# Autodesk Inventor assembly: controller
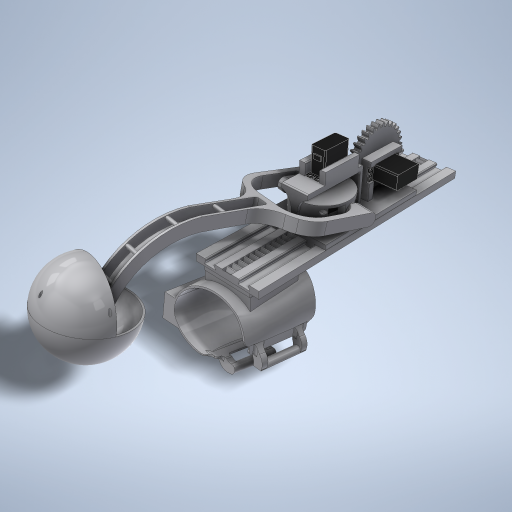
[picture p0: Inventor's stored thumbnail of the model, 512x512]
Saved by Autodesk Inventor 2023 (Build 270158000, 158)
## iProperties
Created: 2024-09-29
Part Number: controller
Document SubType Name: Assembly
Designer: dennis
Author: dennis
## Documents named in this file (15)
- E:\files\controller_v2\final\controller_backup.iam
- E:\files\controller_v2\final\bangle.ipt
- E:\files\controller_v2\final\bangle_ rail_connector.ipt
- E:\files\controller_v2\final\rail.ipt
- rail.ipt
- E:\files\controller_v2\final\carriage.ipt
- E:\files\controller_v2\final\servo_alzrc_ds452mg.ipt
- E:\files\controller_v2\final\servo_horn.ipt
- E:\files\controller_v2\final\gear.ipt
- E:\files\controller_v2\final\ballbearing_servo_mount_swing_axis.ipt
- E:\files\controller_v2\final\servo_mount_swing_axis.ipt
- E:\files\controller_v2\final\ballbearing_pivot_axis.ipt
- E:\files\controller_v2\final\lever.ipt
- E:\files\controller_v2\final\end_effector_halfball.ipt
- E:\files\controller_v2\final\end_effector_quarterball.ipt
## Components (17 placed, 13 different names)
1. bangle_ rail_connector:1 — Slider:1, Rigid:1
2. bangle:1 — Slider:1
3. rail:1 — Rigid:1, Slider:2
4. carriage:1 — Slider:2, Rigid:2, Rotation/Translation:1, Rotation/Translation:2, Rotational:3, Rigid:3
5. servo_alzrc_ds452mg:1 — Rigid:2, Rotational:1
6. servo_horn:1 — Rotational:1, Rotation/Translation:1, Rotational:2
7. gear:1 — Rotational:2, Rotation/Translation:2
8. ballbearing_servo_mount_swing_axis:1 — Rotational:3
9. servo_alzrc_ds452mg:2 — Rigid:3, Rotational:4
10. servo_horn:2 — Rotational:4, Rigid:6
11. servo_mount_swing_axis:1 — Rigid:6, Rigid:7, Rigid:8
12. ballbearing_pivot_axis:1 — Rigid:7
13. servo_alzrc_ds452mg:3 — Rigid:8, Rotational:5
14. servo_horn:3 — Rotational:5, Rigid:9
15. lever:1 — Rigid:9, Rigid:10
16. end_effector_quarterball:1 — Rigid:10, Rigid:11
17. end_effector_halfball:1 — Rigid:11
## Relationships (18: WeldJoint 9, RevoluteJoint 5, TranslationJoint 2, RelateRotateTranslate 2)
- Slider:1 [TranslationJoint]: bangle_ rail_connector:1 ↔ bangle:1
- Rigid:1 [WeldJoint]: bangle_ rail_connector:1 ↔ rail:1
- Slider:2 [TranslationJoint]: rail:1 ↔ carriage:1
- Rigid:2 [WeldJoint]: carriage:1 ↔ servo_alzrc_ds452mg:1
- Rotational:1 [RevoluteJoint]: servo_alzrc_ds452mg:1 ↔ servo_horn:1
- Rotation/Translation:1 [RelateRotateTranslate] (160 mm): carriage:1 ↔ servo_horn:1
- Rotational:2 [RevoluteJoint]: servo_horn:1 ↔ gear:1
- Rotation/Translation:2 [RelateRotateTranslate] (160 mm): carriage:1 ↔ gear:1
- Rotational:3 [RevoluteJoint]: carriage:1 ↔ ballbearing_servo_mount_swing_axis:1
- Rigid:3 [WeldJoint]: carriage:1 ↔ servo_alzrc_ds452mg:2
- Rotational:4 [RevoluteJoint]: servo_alzrc_ds452mg:2 ↔ servo_horn:2
- Rigid:6 [WeldJoint]: servo_horn:2 ↔ servo_mount_swing_axis:1
- Rigid:7 [WeldJoint]: servo_mount_swing_axis:1 ↔ ballbearing_pivot_axis:1
- Rigid:8 [WeldJoint]: servo_mount_swing_axis:1 ↔ servo_alzrc_ds452mg:3
- Rotational:5 [RevoluteJoint]: servo_alzrc_ds452mg:3 ↔ servo_horn:3
- Rigid:9 [WeldJoint]: servo_horn:3 ↔ lever:1
- Rigid:10 [WeldJoint]: lever:1 ↔ end_effector_quarterball:1
- Rigid:11 [WeldJoint]: end_effector_quarterball:1 ↔ end_effector_halfball:1
